# Autodesk Inventor assembly: ThumbMiddlePhalanx
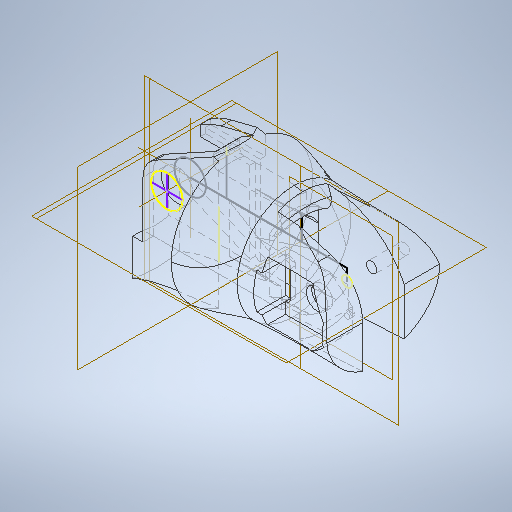
[picture p0: Inventor's stored thumbnail of the model, 512x512]
Saved by Autodesk Inventor 2025.1 (Build 291241000, 241)
## iProperties
Created: 2025-06-06
Part Number: ThumbMiddlePhalanx
Document SubType Name: Assembly
Designer: Alexander
Author: Alexander
## Documents named in this file (3)
- D:\Repositorios_Politecnica\Handi-EPN\CAD\Sim Models\ThumbMiddlePhalanx.iam
- D:\Repositorios_Politecnica\Handi-EPN\CAD\thumb\IP - DTH R.ipt
- D:\Repositorios_Politecnica\Handi-EPN\CAD\thumb\IP - P MainTH R.ipt
## Components (2 placed, 2 different names)
1. IP - DTH R:1 — Mate:1, Flush:3, Flush:4
2. IP - P MainTH R:1 — Mate:1, Flush:3, Flush:4, Mate:2, Mate:3, Mate:4
## Relationships (6: Mate 4, Flush 2)
- Mate:1: IP - DTH R:1 ↔ IP - P MainTH R:1
- Flush:3: IP - DTH R:1 ↔ IP - P MainTH R:1
- Flush:4 (-2.9 mm): IP - DTH R:1 ↔ IP - P MainTH R:1
- Mate:2: IP - P MainTH R:1
- Mate:3: IP - P MainTH R:1
- Mate:4: IP - P MainTH R:1
